# Autodesk Inventor assembly: ShoulderRedesign
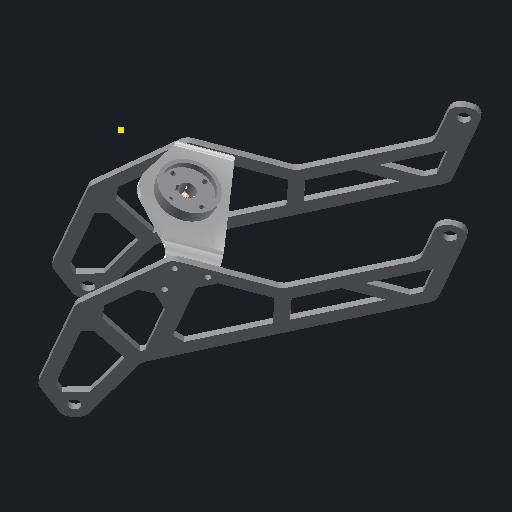
[picture p0: Inventor's stored thumbnail of the model, 512x512]
Saved by Autodesk Inventor 2025.2 (Build 292293000, 293)
## iProperties
Created: 2020-03-24
Part Number: ShoulderRedesign
Document SubType Name: Assembly
Designer: valer
Mass: 383.584 g
Surface Area: 442.479 cm^2
Volume: 56.5483 cm^3
Density: 6.7833 g/cm^3
Author: valer
## Documents named in this file (5)
- C:\Users\valer\Desktop\str1ker\cad\ShoulderRedesign.iam
- C:\Users\valer\Desktop\str1ker\cad\UpperArmBracketBase.ipt
- C:\Users\valer\Desktop\str1ker\cad\ShoulderBoundingBox.ipt
- C:\Users\valer\Desktop\str1ker\cad\ShoulderHub.ipt
- C:\Users\valer\Desktop\str1ker\cad\ShoulderBracketRedesign.ipt
## Components (5 placed, 4 different names)
1. UpperArmBracketBase:1 — Angle:2, Angle:4, Mate:394, Mate:395, Mate:396, Mate:397, Mate:398, Mate:399, Mate:400, Mate:401, Mate:402
2. ShoulderBoundingBox:1 — Mate:393, Angle:4
3. ShoulderHub:1 — Mate:394, Mate:395, Mate:396
4. ShoulderBracketRedesign:1 — Mate:397, Mate:398, Mate:399
5. ShoulderBracketRedesign:2 — Mate:400, Mate:401, Mate:402
## Relationships (12: Mate 10, Angle 2)
- Angle:2 (0 deg): UpperArmBracketBase:1
- Mate:393: ShoulderBoundingBox:1
- Angle:4 (0 deg): UpperArmBracketBase:1 ↔ ShoulderBoundingBox:1
- Mate:394: UpperArmBracketBase:1 ↔ ShoulderHub:1
- Mate:395: UpperArmBracketBase:1 ↔ ShoulderHub:1
- Mate:396: UpperArmBracketBase:1 ↔ ShoulderHub:1
- Mate:397: UpperArmBracketBase:1 ↔ ShoulderBracketRedesign:1
- Mate:398: UpperArmBracketBase:1 ↔ ShoulderBracketRedesign:1
- Mate:399: UpperArmBracketBase:1 ↔ ShoulderBracketRedesign:1
- Mate:400: UpperArmBracketBase:1 ↔ ShoulderBracketRedesign:2
- Mate:401: UpperArmBracketBase:1 ↔ ShoulderBracketRedesign:2
- Mate:402: UpperArmBracketBase:1 ↔ ShoulderBracketRedesign:2
